# Autodesk Inventor assembly: MG-Rolle
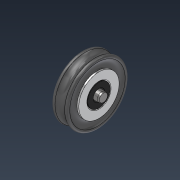
[picture p0: Inventor's stored thumbnail of the model, 180x180]
Saved by Autodesk Inventor 2022.1 (Build 261234020, 234B)
## iProperties
Part Number: MG-Rolle
Material: Generisch
Document SubType Name: Assembly
Designer: rYan
Mass: 1.3472 g
Surface Area: 13.7675 cm^2
Volume: 0.879852 cm^3
Density: 1.53117 g/cm^3
Author: rYan
## Documents named in this file (6)
- D:\TIGERsGIT\Hardware\mechanik\2020\Inventor\Robot\Drive Train\MG-Rolle.iam
- D:\TIGERsGIT\Hardware\mechanik\2020\Inventor\Robot\Drive Train\Rolle.ipt
- D:\TIGERsGIT\Hardware\mechanik\2020\Inventor\Purchased Parts\X-Ring 5.94x3.53.ipt
- D:\TIGERsGIT\Hardware\mechanik\2020\Inventor\Purchased Parts\O-Ring 6x4.0.ipt
- D:\TIGERsGIT\Hardware\mechanik\2020\Inventor\Purchased Parts\Gleitlager MSM-0205-02.ipt
- D:\TIGERsGIT\Hardware\mechanik\2020\Inventor\Inhaltscenter\de-DE\ISO 2338(2)\ISO 2338 - 2 m6 x 6.ipt
## Components (6 placed, 5 different names)
1. X-Ring 5.94x3.53:1 — Passend:7, Fluchtend:2
2. Rolle:1 — Passend:12, Passend:13, Einfügen:1, Einfügen:2
3. ISO 2338 2 m6 x 6:1
4. O-Ring 6x4.0:1 — Passend:15, Fluchtend:7
5. Gleitlager MSM-0205-02:1 — Einfügen:1
6. Gleitlager MSM-0205-02:2 — Einfügen:2
## Relationships (11: Mate 5, Flush 4, Insert 2)
- Passend:7 [Mate]: X-Ring 5.94x3.53:1
- Fluchtend:2 [Flush]: X-Ring 5.94x3.53:1
- Fluchtend:4 [Flush] (-6.8 mm)
- Passend:12 [Mate]: Rolle:1
- Passend:13 [Mate]: Rolle:1
- [Mate]: Rolle:1 ↔ ISO 2338 2 m6 x 6:1
- [Flush] (-3 mm): ISO 2338 2 m6 x 6:1
- Passend:15 [Mate]: O-Ring 6x4.0:1
- Fluchtend:7 [Flush]: O-Ring 6x4.0:1
- Einfügen:1 [Insert]: Rolle:1 ↔ Gleitlager MSM-0205-02:1
- Einfügen:2 [Insert]: Rolle:1 ↔ Gleitlager MSM-0205-02:2
